# Autodesk Inventor assembly: soccer_assembly
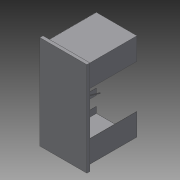
[picture p0: Inventor's stored thumbnail of the model, 180x180]
Saved by Autodesk Inventor 2015 SP1 (Build 190203100, 203)
## iProperties
Created: 2018-04-13
Part Number: soccer_assembly
Document SubType Name: Assembly
Designer: 407642
Author: 407642
## Documents named in this file (5)
- H:\2017 CARDERROCK\soccer_assembly.iam
- H:\2017 CARDERROCK\soccer_goal.ipj.ipt
- H:\2017 CARDERROCK\sonar.ipt
- H:\2017 CARDERROCK\button.ipt
- H:\2017 CARDERROCK\limit_switch.ipt
## Components (5 placed, 4 different names)
1. soccer_goal.ipj:1 — Mate:1, Mate:2, Mate:3, Mate:4, Mate:5, Mate:6, Mate:7, Flush:1, Mate:8, Mate:9, Flush:2, Flush:3
2. sonar:1 — Mate:4, Mate:5, Mate:6
3. sonar:2 — Mate:1, Mate:2, Mate:3
4. button:1 — Mate:7, Flush:1, Mate:8
5. limit_switch:1 — Mate:9, Flush:2, Flush:3
## Relationships (12: Mate 9, Flush 3)
- Mate:1: soccer_goal.ipj:1 ↔ sonar:2
- Mate:2 (4 mm): soccer_goal.ipj:1 ↔ sonar:2
- Mate:3 (5 mm): soccer_goal.ipj:1 ↔ sonar:2
- Mate:4: soccer_goal.ipj:1 ↔ sonar:1
- Mate:5 (5 mm): soccer_goal.ipj:1 ↔ sonar:1
- Mate:6 (4 mm): soccer_goal.ipj:1 ↔ sonar:1
- Mate:7: soccer_goal.ipj:1 ↔ button:1
- Flush:1 (20 mm): soccer_goal.ipj:1 ↔ button:1
- Mate:8 (55 mm): soccer_goal.ipj:1 ↔ button:1
- Mate:9: soccer_goal.ipj:1 ↔ limit_switch:1
- Flush:2 (-13 mm): soccer_goal.ipj:1 ↔ limit_switch:1
- Flush:3 (40 mm): soccer_goal.ipj:1 ↔ limit_switch:1
